# Autodesk Inventor assembly: Robot Chassis 2014
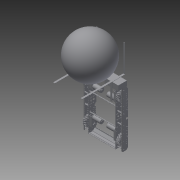
[picture p0: Inventor's stored thumbnail of the model, 180x180]
Saved by Autodesk Inventor 2013 (Build 170138000, 138)
## iProperties
Created: 2014-01-08
Part Number: Robot Chassis 2014
Document SubType Name: Assembly
Designer: 300593
Translation Standard: STEP AP203
FileName: AM14U Long and AM14U Wide.STEP
PreProcessor: SolidWorks 2010
PostProcessor: Build: 138, Release: 2013 RTM - Date: Thu 03/01/2012
Sent Units: inch
Uncertainty: 1e-05
Author: 300593
## Documents named in this file (9)
- E:\Robotics\FRC\2014\CAD\Frame\Robot Chassis 2014.iam
- E:\Robotics\FRC\2014\CAD\Frame\AM14U Long.iam
- E:\Robotics\FRC\2014\CAD\Frame\Left-6-inch-HD-Mecanum-Wheel.iam
- E:\Robotics\FRC\2014\CAD\Frame\Right-6-inch-HD-Mecanum-Wheel.iam
- E:\Robotics\FRC\2014\CAD\Frame\Toughbox-nano-hex-asm.iam
- E:\Robotics\FRC\2014\CAD\Additions\BumperFront.ipt
- E:\Robotics\FRC\2014\CAD\Additions\ArmTest.ipt
- E:\Robotics\FRC\2014\CAD\Additions\Ball.ipt
- E:\Robotics\FRC\2014\CAD\Additions\TemporaryBlock.ipt
## Components (14 placed, 8 different names)
1. AM14U Long:1 [sub-assembly] — Mate:1, Mate:2, Mate:3, Mate:4, Mate:5, Mate:6, Mate:7, Mate:8, Mate:9, Mate:10, Mate:11, Mate:12, Mate:17, Mate:18, Mate:19, Mate:20, Flush:1, Flush:8, Flush:9
2. Left-6-inch-HD-Mecanum-Wheel:1 [sub-assembly] — Mate:16, Mate:17
3. Left-6-inch-HD-Mecanum-Wheel:2 [sub-assembly] — Mate:14, Mate:20
4. Right-6-inch-HD-Mecanum-Wheel:1 [sub-assembly] — Mate:13, Mate:19
5. Right-6-inch-HD-Mecanum-Wheel:2 [sub-assembly] — Mate:15, Mate:18
6. Toughbox-nano-hex-asm:1 [sub-assembly] — Mate:7, Mate:10, Mate:12, Mate:13
7. Toughbox-nano-hex-asm:2 [sub-assembly] — Mate:8, Mate:9, Mate:11, Mate:14, Flush:10
8. Toughbox-nano-hex-asm:3 [sub-assembly] — Mate:4, Mate:5, Mate:6, Mate:15
9. Toughbox-nano-hex-asm:4 [sub-assembly] — Mate:1, Mate:2, Mate:3, Mate:16
10. BumperFront:1 — Flush:1, Flush:2, Flush:5, Flush:6, Flush:7
11. ArmTest:1 — Flush:2, Flush:3, Flush:4, Mate:21, Flush:7, Mate:22, Flush:11
12. ArmTest:2 — Flush:3, Flush:4, Mate:21
13. Ball:1 — Flush:5, Flush:6
14. TemporaryBlock:1 — Flush:8, Flush:9, Mate:22, Flush:10, Flush:11
## Relationships (33: Mate 22, Flush 11)
- Mate:1: AM14U Long:1 ↔ Toughbox-nano-hex-asm:4
- Mate:2: AM14U Long:1 ↔ Toughbox-nano-hex-asm:4
- Mate:3: AM14U Long:1 ↔ Toughbox-nano-hex-asm:4
- Mate:4: AM14U Long:1 ↔ Toughbox-nano-hex-asm:3
- Mate:5: AM14U Long:1 ↔ Toughbox-nano-hex-asm:3
- Mate:6: AM14U Long:1 ↔ Toughbox-nano-hex-asm:3
- Mate:7: AM14U Long:1 ↔ Toughbox-nano-hex-asm:1
- Mate:8: AM14U Long:1 ↔ Toughbox-nano-hex-asm:2
- Mate:9: AM14U Long:1 ↔ Toughbox-nano-hex-asm:2
- Mate:10: AM14U Long:1 ↔ Toughbox-nano-hex-asm:1
- Mate:11: AM14U Long:1 ↔ Toughbox-nano-hex-asm:2
- Mate:12: AM14U Long:1 ↔ Toughbox-nano-hex-asm:1
- Mate:13: Right-6-inch-HD-Mecanum-Wheel:1 ↔ Toughbox-nano-hex-asm:1
- Mate:14: Left-6-inch-HD-Mecanum-Wheel:2 ↔ Toughbox-nano-hex-asm:2
- Mate:15: Right-6-inch-HD-Mecanum-Wheel:2 ↔ Toughbox-nano-hex-asm:3
- Mate:16: Left-6-inch-HD-Mecanum-Wheel:1 ↔ Toughbox-nano-hex-asm:4
- Mate:17 (19.3294 mm): AM14U Long:1 ↔ Left-6-inch-HD-Mecanum-Wheel:1
- Mate:18 (19.3294 mm): AM14U Long:1 ↔ Right-6-inch-HD-Mecanum-Wheel:2
- Mate:19 (19.3294 mm): AM14U Long:1 ↔ Right-6-inch-HD-Mecanum-Wheel:1
- Mate:20 (19.3294 mm): AM14U Long:1 ↔ Left-6-inch-HD-Mecanum-Wheel:2
- Flush:1: AM14U Long:1 ↔ BumperFront:1
- Flush:2: BumperFront:1 ↔ ArmTest:1
- Flush:3: ArmTest:1 ↔ ArmTest:2
- Flush:4: ArmTest:1 ↔ ArmTest:2
- Mate:21 (381 mm): ArmTest:1 ↔ ArmTest:2
- Flush:5: BumperFront:1 ↔ Ball:1
- Flush:6 (304.8 mm): BumperFront:1 ↔ Ball:1
- Flush:7 (76.2 mm): BumperFront:1 ↔ ArmTest:1
- Flush:8: AM14U Long:1 ↔ TemporaryBlock:1
- Flush:9: AM14U Long:1 ↔ TemporaryBlock:1
- Mate:22: ArmTest:1 ↔ TemporaryBlock:1
- Flush:10 (60.325 mm): Toughbox-nano-hex-asm:2 ↔ TemporaryBlock:1
- Flush:11 (12.7 mm): ArmTest:1 ↔ TemporaryBlock:1
